# Autodesk Inventor assembly: Assembly3
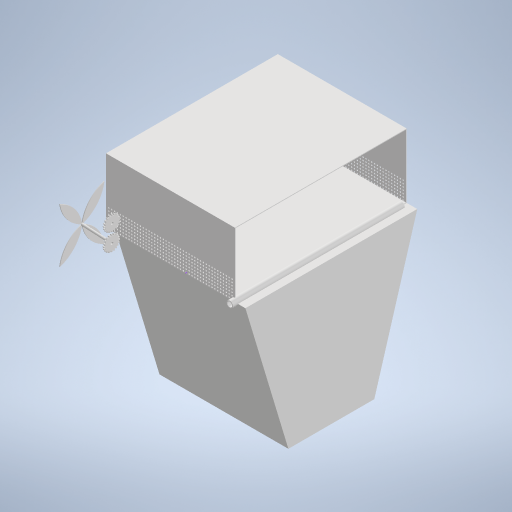
[picture p0: Inventor's stored thumbnail of the model, 512x512]
Saved by Autodesk Inventor 2024 (Build 280153000, 153)
## iProperties
Created: 2024-09-04
Part Number: Assembly3
Document SubType Name: Assembly
Designer: srira
Author: srira
## Documents named in this file (6)
- C:\Users\srira\Documents\IITGN\3rd year\Sem5\ES408\Tentative Model\Assembly3.iam
- C:\Users\srira\Documents\IITGN\3rd year\Sem5\ES408\Tentative Model\Dustbin Body.ipt
- C:\Users\srira\Documents\IITGN\3rd year\Sem5\ES408\Tentative Model\Ger.ipt
- C:\Users\srira\Documents\IITGN\3rd year\Sem5\ES408\Tentative Model\ranpro.ipt
- C:\Users\srira\Documents\IITGN\3rd year\Sem5\ES408\Tentative Model\Roller.ipt
- C:\Users\srira\Documents\IITGN\3rd year\Sem5\ES408\Tentative Model\Trap.ipt
## Components (9 placed, 5 different names)
1. Dustbin Body:1 — Mate:6, Mate:9, Mate:10
2. Roller:1 — Mate:6
3. Ger:1 — Mate:7
4. Ger:2 — Mate:8
5. Ger:3 — Mate:8, Insert:2
6. Ger:4 — Mate:7, Insert:1
7. ranpro:1 — Insert:2
8. ranpro:2 — Insert:1
9. Trap:1 — Mate:9, Mate:10
## Relationships (7: Mate 5, Insert 2)
- Mate:6: Dustbin Body:1 ↔ Roller:1
- Mate:7: Ger:1 ↔ Ger:4
- Insert:1: Ger:4 ↔ ranpro:2
- Mate:8: Ger:2 ↔ Ger:3
- Insert:2: Ger:3 ↔ ranpro:1
- Mate:9: Dustbin Body:1 ↔ Trap:1
- Mate:10: Dustbin Body:1 ↔ Trap:1
